# Autodesk Inventor assembly: Ryan final assembley
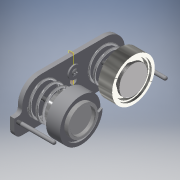
[picture p0: Inventor's stored thumbnail of the model, 180x180]
Saved by Autodesk Inventor 2017.3 (Build 213256000, 256)
## iProperties
Created: 2017-04-26
Part Number: Ryan final assembley
Document SubType Name: Assembly
Designer: 196918
Author: 196918
## Documents named in this file (15)
- C:\Users\rbibb\Desktop\8.1\Ryan final assembley.iam
- C:\Users\rbibb\Desktop\8.1\Base plate.ipt
- C:\Users\rbibb\Desktop\8.1\lever arm.ipt
- C:\Users\rbibb\Desktop\8.1\lower die 1 center.ipt
- C:\Users\rbibb\Desktop\8.1\lower die 1 outer ring.ipt
- C:\Users\rbibb\Desktop\8.1\Lower die 2 center.ipt
- C:\Users\rbibb\Desktop\8.1\Lower die 2 oweder ring.ipt
- C:\Users\rbibb\Desktop\8.1\lower die 2 spacer.ipt
- C:\Users\rbibb\Desktop\8.1\tiny screw.ipt
- C:\Users\rbibb\Desktop\8.1\Waher.ipt
- C:\Users\rbibb\Desktop\8.1\lever arm_MIR.ipt
- C:\Users\rbibb\Desktop\8.1\Bottom Die Spring 1.ipt
- C:\Users\rbibb\Desktop\8.1\Bottom Die Spring 1_MIR.ipt
- C:\Users\rbibb\Desktop\8.1\screw.ipt
- C:\Users\rbibb\Desktop\8.1\screw_MIR.ipt
## Components (14 placed, 14 different names)
1. Base plate:1 — Rigid:1, Mate:1, Angle:1, Mate:2, Angle:2, Rotational:6, Rotational:9, Rotational:10
2. lever arm:1 — Rigid:1
3. lower die 1 center:1 — Rotational:5
4. lower die 1 outer ring:1 — Rotational:5
5. Lower die 2 center:1 — Rotational:3
6. Lower die 2 oweder ring:1 — Rotational:2, Rotational:3
7. lower die 2 spacer:1 — Rotational:2
8. tiny screw:1 — Rotational:6, Rotational:7
9. Waher:1 — Rotational:7
10. lever arm_MIR:2
11. Bottom Die Spring 1:1 — Rotational:9
12. Bottom Die Spring 1_MIR:1
13. screw:1 — Rotational:10
14. screw_MIR:1
## Relationships (13: RevoluteJoint 7, Mate 2, Angle 2, WeldJoint 1, Symmetry 1)
- Rigid:1 [WeldJoint]: Base plate:1 ↔ lever arm:1
- Mate:1: Base plate:1
- Angle:1 (0 deg): Base plate:1
- Mate:2: Base plate:1
- Angle:2 (0 deg): Base plate:1
- Symmetry:1
- Rotational:2 [RevoluteJoint]: Lower die 2 oweder ring:1 ↔ lower die 2 spacer:1
- Rotational:3 [RevoluteJoint]: Lower die 2 center:1 ↔ Lower die 2 oweder ring:1
- Rotational:5 [RevoluteJoint]: lower die 1 center:1 ↔ lower die 1 outer ring:1
- Rotational:6 [RevoluteJoint]: Base plate:1 ↔ tiny screw:1
- Rotational:7 [RevoluteJoint]: tiny screw:1 ↔ Waher:1
- Rotational:9 [RevoluteJoint]: Base plate:1 ↔ Bottom Die Spring 1:1
- Rotational:10 [RevoluteJoint]: Base plate:1 ↔ screw:1
